# Autodesk Inventor assembly: gantry
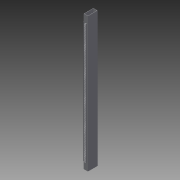
[picture p0: Inventor's stored thumbnail of the model, 180x180]
Saved by Autodesk Inventor 2013 (Build 170138000, 138)
## iProperties
Created: 2012-11-30
Part Number: gantry
Document SubType Name: Assembly
Designer: istvan.burbank
Author: istvan.burbank
## Documents named in this file (5)
- D:\GitHub\Crown-Fire\CAD\Frame\Gantry\gantry.iam
- D:\GitHub\Crown-Fire\CAD\Frame\Gantry\gantryFrame.ipt
- D:\GitHub\Crown-Fire\CAD\Frame\Linear Motion\rack-x.ipt
- D:\GitHub\Crown-Fire\CAD\Frame\Linear Motion\vee-track-x.ipt
- D:\GitHub\Crown-Fire\CAD\Templates\squareTube1.75x4.ipt
## Components (4 placed, 3 different names)
1. gantryFrame:1 — Mate:1, Angle:1, Flush:2, Flush:3, Mate:2, Mate:3, Mate:4, Mate:5
2. rack-x:1 — Mate:1, Angle:1, Flush:2, Flush:3, Flush:4, Flush:5
3. vee-track-x:1 — Mate:2, Mate:5, Flush:4
4. vee-track-x:2 — Mate:3, Mate:4, Flush:5
## Relationships (10: Mate 5, Flush 4, Angle 1)
- Mate:1: gantryFrame:1 ↔ rack-x:1
- Angle:1 (0 deg): gantryFrame:1 ↔ rack-x:1
- Flush:2 (-76.2 mm): gantryFrame:1 ↔ rack-x:1
- Flush:3 (-12.7 mm): gantryFrame:1 ↔ rack-x:1
- Mate:2: gantryFrame:1 ↔ vee-track-x:1
- Mate:3: gantryFrame:1 ↔ vee-track-x:2
- Mate:4: gantryFrame:1 ↔ vee-track-x:2
- Mate:5: gantryFrame:1 ↔ vee-track-x:1
- Flush:4: rack-x:1 ↔ vee-track-x:1
- Flush:5: rack-x:1 ↔ vee-track-x:2
